# Autodesk Inventor assembly: rightHalfOfFrameV03_MIR
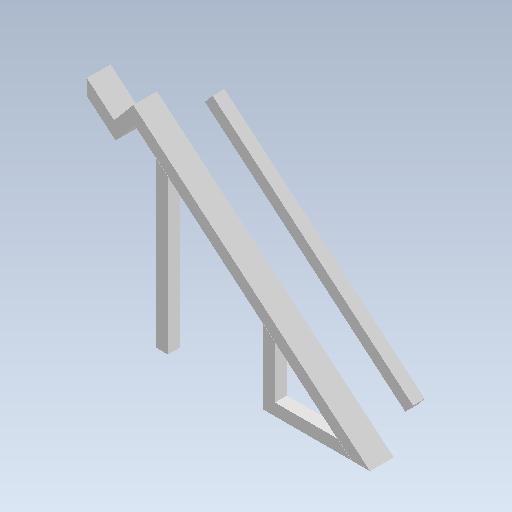
[picture p0: Inventor's stored thumbnail of the model, 512x512]
Saved by Autodesk Inventor 2020.2 (Build 242310000, 310)
## iProperties
Created: 2020-02-22
Part Number: rightHalfOfFrameV03_MIR
Document SubType Name: Assembly
Designer: robst
Author: robst
## Documents named in this file (4)
- C:\git\CAD-Development\robSteele\2020LongRobotBase\rightHalfOfFrameV03_MIR.iam
- C:\git\CAD-Development\robSteele\2020LongRobotBase\newFrame1x1V03_MIR.ipt
- C:\git\CAD-Development\robSteele\2020LongRobotBase\newFrame1x2piecsV03_MIR.ipt
- C:\git\CAD-Development\robSteele\2020LongRobotBase\newPullyV03_MIR.ipt
## Components (3 placed, 3 different names)
1. newFrame1x1V03_MIR:1 — Flush:2, Flush:1, Mate:1
2. newFrame1x2piecsV03_MIR:1 — Flush:2, Flush:1, Mate:1, Mate:2, Flush:3
3. newPullyV03_MIR:1 — Mate:2, Flush:3
## Relationships (5: Mate 3, Flush 2)
- Flush:2: newFrame1x1V03_MIR:1 ↔ newFrame1x2piecsV03_MIR:1
- Flush:1: newFrame1x1V03_MIR:1 ↔ newFrame1x2piecsV03_MIR:1
- Mate:1: newFrame1x1V03_MIR:1 ↔ newFrame1x2piecsV03_MIR:1
- Mate:2 (127 mm): newFrame1x2piecsV03_MIR:1 ↔ newPullyV03_MIR:1
- Flush:3 [Mate] (63.5 mm): newFrame1x2piecsV03_MIR:1 ↔ newPullyV03_MIR:1
